# Autodesk Inventor assembly: SM1_scanlensholder_on_mount
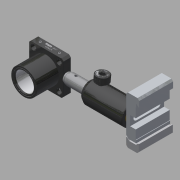
[picture p0: Inventor's stored thumbnail of the model, 180x180]
Saved by Autodesk Inventor 2018 (Build 220112000, 112)
## iProperties
Created: 2018-09-24
Part Number: SM1_scanlensholder_on_mount
Document SubType Name: Assembly
Designer: Robert Campbell
Author: Robert Campbell
## Documents named in this file (6)
- X:\home\work\Documents\MF_BenchOptics\CAD_files\SM1_scanlensholder_on_mount.iam
- X:\home\work\Documents\MF_BenchOptics\CAD_files\TR50_M-Solidworks.ipt
- X:\home\work\Documents\MF_BenchOptics\CAD_files\PH50_M-Solidworks.ipt
- X:\home\work\Documents\MF_BenchOptics\CAD_files\XT66C4-Step.ipt
- W:\home\work\Documents\MF_BenchOptics\CAD_files\SM1L10-Solidworks.ipt
- W:\home\work\Documents\MF_BenchOptics\CAD_files\CP02_M-Solidworks.ipt
## Components (5 placed, 5 different names)
1. TR50_M-Solidworks:1 — Mate:1, Mate:2, Mate:6, Mate:9, Mate:10
2. PH50_M-Solidworks:1 — Mate:1, Mate:2, Mate:5
3. XT66C4-Step:1 — Mate:5, Mate:6, Angle:1
4. SM1L10-Solidworks:1 — Mate:7, Mate:8
5. CP02_M-Solidworks:1 — Mate:7, Mate:8, Mate:9, Mate:10, Angle:1
## Relationships (9: Mate 8, Angle 1)
- Mate:1: TR50_M-Solidworks:1 ↔ PH50_M-Solidworks:1
- Mate:2 (20 mm): TR50_M-Solidworks:1 ↔ PH50_M-Solidworks:1
- Mate:5: PH50_M-Solidworks:1 ↔ XT66C4-Step:1
- Mate:6: TR50_M-Solidworks:1 ↔ XT66C4-Step:1
- Mate:7: SM1L10-Solidworks:1 ↔ CP02_M-Solidworks:1
- Mate:8: SM1L10-Solidworks:1 ↔ CP02_M-Solidworks:1
- Mate:9: TR50_M-Solidworks:1 ↔ CP02_M-Solidworks:1
- Mate:10: TR50_M-Solidworks:1 ↔ CP02_M-Solidworks:1
- Angle:1 (0 deg): XT66C4-Step:1 ↔ CP02_M-Solidworks:1
